# Autodesk Inventor assembly: PI holder
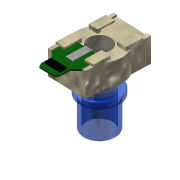
[picture p0: Inventor's stored thumbnail of the model, 180x180]
Saved by Autodesk Inventor 2014 (Build 180170000, 170)
## iProperties
Created: 2016-07-07
Part Number: PI holder
Document SubType Name: Assembly
Designer: Camilo
Author: Camilo
## Documents named in this file (6)
- Z:\Github\AgingTests\3D parts\PI holder\PI holder.iam
- Z:\Github\AgingTests\3D parts\ECoG holder\flaskPort.ipt
- Z:\Github\AgingTests\3D parts\PI holder\FalconTube15mL.ipt
- Z:\Github\AgingTests\3D parts\PI holder\PI_holder.ipt
- Z:\Github\AgingTests\3D parts\PI holder\WirebondAdapter.ipt
- Z:\Github\AgingTests\3D parts\PI holder\PIElectrodes.ipt
## Components (5 placed, 5 different names)
1. flaskPort:1 — Flush:1, Flush:2, Flush:3, Mate:1, Flush:4
2. FalconTube15mL:1 — Mate:1, Flush:4, Flush:5, Flush:6
3. PI_holder:1 — Flush:6, Mate:2, Tangent:1, Mate:3
4. WirebondAdapter:1 — Mate:2, Tangent:1, Mate:3, Mate:4, Mate:5, Mate:6
5. PIElectrodes:1 — Mate:4, Mate:5, Mate:6
## Relationships (13: Flush 6, Mate 6, Tangent 1)
- Flush:1: flaskPort:1
- Flush:2: flaskPort:1
- Flush:3: flaskPort:1
- Mate:1: flaskPort:1 ↔ FalconTube15mL:1
- Flush:4 (-2 mm): flaskPort:1 ↔ FalconTube15mL:1
- Flush:5: FalconTube15mL:1
- Flush:6: FalconTube15mL:1 ↔ PI_holder:1
- Mate:2: PI_holder:1 ↔ WirebondAdapter:1
- Tangent:1: PI_holder:1 ↔ WirebondAdapter:1
- Mate:3: PI_holder:1 ↔ WirebondAdapter:1
- Mate:4: WirebondAdapter:1 ↔ PIElectrodes:1
- Mate:5 (1 mm): WirebondAdapter:1 ↔ PIElectrodes:1
- Mate:6: WirebondAdapter:1 ↔ PIElectrodes:1
